# Autodesk Inventor assembly: Z axis motor mount sub-assembly
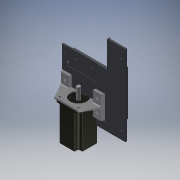
[picture p0: Inventor's stored thumbnail of the model, 180x180]
Saved by Autodesk Inventor 2018 (Build 220112000, 112)
## iProperties
Created: 2018-03-20
Part Number: Z axis motor mount sub-assembly
Document SubType Name: Assembly
Designer: M224826
Author: M224826
## Documents named in this file (4)
- C:\Users\M224826\Documents\GitHub\CNC-Lathe-CAD\Lathe with updated parts (LATEST of 20 06 17)\Z axis motor mount sub-assembly.iam
- C:\Users\M224826\Documents\GitHub\CNC-Lathe-CAD\Lathe with updated parts (LATEST of 20 06 17)\Motor Support Fin.ipt
- C:\Users\M224826\Documents\GitHub\CNC-Lathe-CAD\Lathe with updated parts (LATEST of 20 06 17)\SUPPORT MAIN FRAME MOTOR-BALL SCREW-REV-B.ipt
- C:\Users\M224826\Documents\GitHub\CNC-Lathe-CAD\Lathe with updated parts (LATEST of 20 06 17)\Servo Motor\Servo Motor.iam
## Components (3 placed, 3 different names)
1. Motor Support Fin:1 — Mate:1, Mate:2, Mate:3, Mate:4, Mate:5, Angle:1
2. SUPPORT MAIN FRAME MOTOR-BALL SCREW-REV-B:1 — Flush:1, Flush:2, Flush:3, Mate:1, Mate:2, Mate:3
3. Servo Motor:1 [sub-assembly] — Mate:4, Mate:5, Angle:1
## Relationships (9: Mate 5, Flush 3, Angle 1)
- Flush:1: SUPPORT MAIN FRAME MOTOR-BALL SCREW-REV-B:1
- Flush:2: SUPPORT MAIN FRAME MOTOR-BALL SCREW-REV-B:1
- Flush:3: SUPPORT MAIN FRAME MOTOR-BALL SCREW-REV-B:1
- Mate:1: Motor Support Fin:1 ↔ SUPPORT MAIN FRAME MOTOR-BALL SCREW-REV-B:1
- Mate:2: Motor Support Fin:1 ↔ SUPPORT MAIN FRAME MOTOR-BALL SCREW-REV-B:1
- Mate:3: Motor Support Fin:1 ↔ SUPPORT MAIN FRAME MOTOR-BALL SCREW-REV-B:1
- Mate:4: Motor Support Fin:1 ↔ Servo Motor:1
- Mate:5: Motor Support Fin:1 ↔ Servo Motor:1
- Angle:1 (0 deg): Motor Support Fin:1 ↔ Servo Motor:1
